# Autodesk Inventor assembly: Updated Gearset MJF Shaft + Carrier
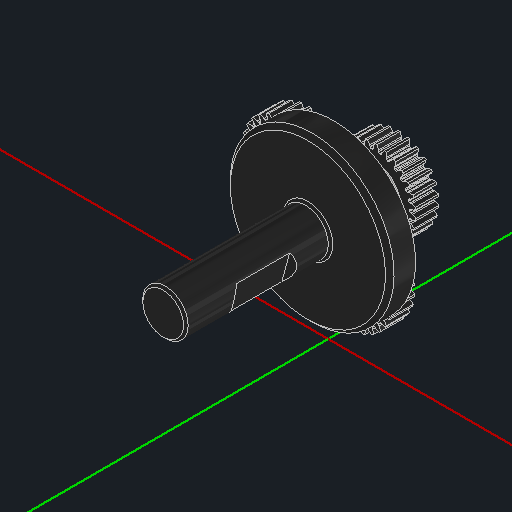
[picture p0: Inventor's stored thumbnail of the model, 512x512]
Saved by Autodesk Inventor 2022.2 (Build 262287010, 287A)
## iProperties
Created: 2022-03-15
Part Number: Updated Gearset MJF Shaft + Carrier
Document SubType Name: Assembly
Designer: sleib
Author: sleib
## Documents named in this file (4)
- C:\Users\sleib\Projekte\Voron-2\CAD\Inventor\Galileo Clockwork\Updated Gearset MJF Shaft + Carrier.iam
- C:\Users\sleib\Projekte\Voron-2\CAD\Inventor\Galileo Clockwork\PlanetSpider_5mm V2.ipt
- C:\Users\sleib\Projekte\Voron-2\CAD\Inventor\Galileo Clockwork\MR95ZZ v1.ipt
- C:\Users\sleib\Projekte\Voron-2\CAD\Inventor\Galileo Clockwork\Spur Gear (27 teeth) 9mm Bearing.ipt
## Components (7 placed, 3 different names)
1. PlanetSpider_5mm V2:1 — Passend:1, Fluchtend:1, Passend:2, Passend:3, Passend:4, Passend:5, Passend:6, Passend:7
2. MR95ZZ v1:1 — Passend:2, Passend:6, Passend:9, Passend:13
3. MR95ZZ v1:2 — Passend:3, Passend:5, Passend:8, Passend:11
4. MR95ZZ v1:3 — Passend:4, Passend:7, Passend:10, Passend:12
5. Spur Gear (27 teeth) 9mm Bearing:1 — Passend:10, Passend:12
6. Spur Gear (27 teeth) 9mm Bearing:2 — Passend:9, Passend:13
7. Spur Gear (27 teeth) 9mm Bearing:3 — Passend:8, Passend:11
## Relationships (14: Mate 13, Flush 1)
- Passend:1 [Mate]: PlanetSpider_5mm V2:1
- Fluchtend:1 [Flush]: PlanetSpider_5mm V2:1
- Passend:2 [Mate]: PlanetSpider_5mm V2:1 ↔ MR95ZZ v1:1
- Passend:3 [Mate]: PlanetSpider_5mm V2:1 ↔ MR95ZZ v1:2
- Passend:4 [Mate]: PlanetSpider_5mm V2:1 ↔ MR95ZZ v1:3
- Passend:5 [Mate]: PlanetSpider_5mm V2:1 ↔ MR95ZZ v1:2
- Passend:6 [Mate]: PlanetSpider_5mm V2:1 ↔ MR95ZZ v1:1
- Passend:7 [Mate]: PlanetSpider_5mm V2:1 ↔ MR95ZZ v1:3
- Passend:8 [Mate]: MR95ZZ v1:2 ↔ Spur Gear (27 teeth) 9mm Bearing:3
- Passend:9 [Mate]: MR95ZZ v1:1 ↔ Spur Gear (27 teeth) 9mm Bearing:2
- Passend:10 [Mate]: MR95ZZ v1:3 ↔ Spur Gear (27 teeth) 9mm Bearing:1
- Passend:11 [Mate]: MR95ZZ v1:2 ↔ Spur Gear (27 teeth) 9mm Bearing:3
- Passend:12 [Mate]: MR95ZZ v1:3 ↔ Spur Gear (27 teeth) 9mm Bearing:1
- Passend:13 [Mate]: MR95ZZ v1:1 ↔ Spur Gear (27 teeth) 9mm Bearing:2
